# Autodesk Inventor assembly: 4inchTire-1111-2017_MIR
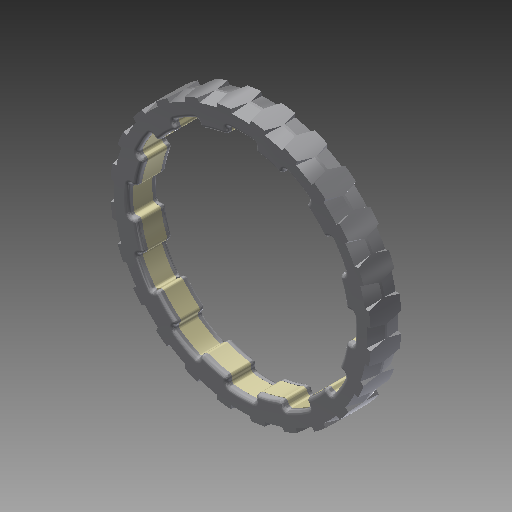
[picture p0: Inventor's stored thumbnail of the model, 512x512]
Saved by Autodesk Inventor 2018 (Build 220112000, 112)
## iProperties
Created: 2013-12-10
Part Number: 4inchTire-1111-2017_MIR
Description: STEP AP214
Document SubType Name: Assembly
Designer: Power Hawks CADD
Mass: 39.854 g
Surface Area: 242.069 cm^2
Volume: 32.2803 cm^3
Density: 1.23462 g/cm^3
Title: 217-2859-STEP.STEP
Revision Number: ANY
Sending System: SolidWorks 2013
Preprocessor: SwSTEP 2.0
## Documents named in this file (3)
- F:\GrabCad\Resources\VEXpro Resources\Wheels\Wheel Parts\4InchTire\4inchTire-1111-2017_MIR.iam
- F:\GrabCad\Resources\VEXpro Resources\Wheels\Wheel Parts\4InchTire\217-2859-001 Rev4_MIR.ipt
- F:\GrabCad\Resources\VEXpro Resources\Wheels\Wheel Parts\4InchTire\217-2859-011 rev3_MIR.ipt
## Components (2 placed, 2 different names)
1. 217-2859-001 Rev4_MIR:1 — Rigid:1
2. 217-2859-011 rev3_MIR:1 — Rigid:1
## Relationships (1: WeldJoint 1)
- Rigid:1 [WeldJoint]: 217-2859-001 Rev4_MIR:1 ↔ 217-2859-011 rev3_MIR:1
